# Autodesk Inventor assembly: Application_openUC2_QBox_2
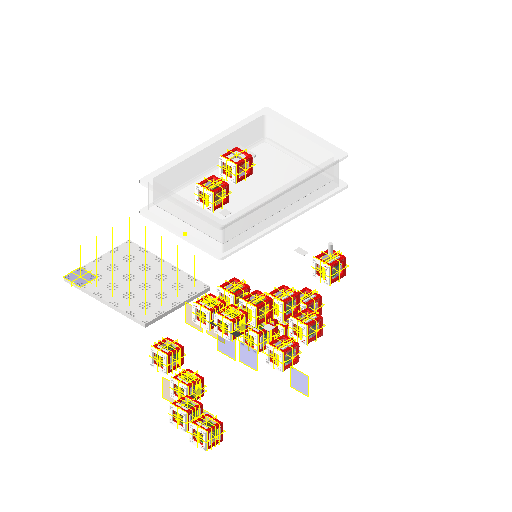
[picture p0: Inventor's stored thumbnail of the model, 512x512]
Saved by Autodesk Inventor 2025.1 (Build 291241020, 241B)
## iProperties
Created: 2022-07-25
Part Number: Application_openUC2_QBox_2
Document SubType Name: Assembly
Designer: diederichbenedict
Mass: 3359.27 g
Surface Area: 10315 cm^2
Volume: 3354.93 cm^3
Density: 1.00129 g/cm^3
Author: diederichbenedict
## Documents named in this file (12)
- C:\Users\diederichbenedict\Dropbox\Dokumente\Promotion\PROJECTS\TechnicalDocs-openUC2-QBox\Production_Files\CAD_Files\INVENTOR\Application_openUC2_QBox_2.iam
- C:\Users\diederichbenedict\Dropbox\Dokumente\Promotion\PROJECTS\TechnicalDocs-openUC2-QBox\Production_Files\CAD_Files\INVENTOR\00_Really_Useful_Box_4l_DinA4_body.ipt
- C:\Users\diederichbenedict\Dropbox\Dokumente\Promotion\PROJECTS\TechnicalDocs-openUC2-QBox\Production_Files\CAD_Files\INVENTOR\Assembly_Cube_v4_Beamsplittercube_20mm.iam
- C:\Users\diederichbenedict\Dropbox\Dokumente\Promotion\PROJECTS\TechnicalDocs-openUC2-QBox\Production_Files\CAD_Files\INVENTOR\Assembly_Cube_v4_Lens.iam
- C:\Users\diederichbenedict\Dropbox\Dokumente\Promotion\PROJECTS\TechnicalDocs-openUC2-QBox\Production_Files\CAD_Files\INVENTOR\Assembly_Cube_v4_KinematicMirror_45°.iam
- C:\Users\diederichbenedict\Dropbox\Dokumente\Promotion\PROJECTS\TechnicalDocs-openUC2-QBox\Production_Files\CAD_Files\INVENTOR\Assembly_Cube_v4_Photosensor.iam
- C:\Users\diederichbenedict\Dropbox\Dokumente\Promotion\PROJECTS\TechnicalDocs-openUC2-QBox\Production_Files\CAD_Files\INVENTOR\Assembly_Cube_v4_polfilter.iam
- C:\Users\diederichbenedict\Dropbox\Dokumente\Promotion\PROJECTS\TechnicalDocs-openUC2-QBox\Production_Files\CAD_Files\INVENTOR\Assembly_Cube_v4_magnet_tshirt.iam
- C:\Users\diederichbenedict\Dropbox\Dokumente\Promotion\PROJECTS\TechnicalDocs-openUC2-QBox\Production_Files\CAD_Files\INVENTOR\Assembly_Cube_v4_slideframe_holder.iam
- C:\Users\diederichbenedict\Dropbox\Dokumente\Promotion\PROJECTS\TechnicalDocs-openUC2-QBox\Production_Files\CAD_Files\INVENTOR\Assembly_Cube_v4_xystage_diamond.iam
- C:\Users\diederichbenedict\Dropbox\Dokumente\Promotion\PROJECTS\TechnicalDocs-openUC2-QBox\Production_Files\CAD_Files\INVENTOR\20_Baseplate_POM_10mm.ipt
- C:\Users\diederichbenedict\Dropbox\Dokumente\Promotion\PROJECTS\TechnicalDocs-openUC2-QBox\Production_Files\CAD_Files\INVENTOR\Assembly_Cube_v4_Laser_v4.iam
## Components (20 placed, 11 different names)
1. 00_Really_Useful_Box_4l_DinA4_body:1 — Mate:12
2. Assembly_Cube_v4_Beamsplittercube_20mm:1 [sub-assembly]
3. Assembly_Cube_v4_Beamsplittercube_20mm:2 [sub-assembly]
4. Assembly_Cube_v4_Beamsplittercube_20mm:4 [sub-assembly]
5. Assembly_Cube_v4_Beamsplittercube_20mm:3 [sub-assembly]
6. Assembly_Cube_v4_KinematicMirror_45°:1 [sub-assembly]
7. Assembly_Cube_v4_KinematicMirror_45°:2 [sub-assembly]
8. Assembly_Cube_v4_KinematicMirror_45°:3 [sub-assembly]
9. Assembly_Cube_v4_polfilter:1 [sub-assembly]
10. Assembly_Cube_v4_polfilter:2 [sub-assembly]
11. Assembly_Cube_v4_magnet_tshirt:1 [sub-assembly]
12. Assembly_Cube_v4_Lens:1 [sub-assembly]
13. Assembly_Cube_v4_Lens:2 [sub-assembly]
14. Assembly_Cube_v4_Lens:3 [sub-assembly]
15. Assembly_Cube_v4_Photosensor:1 [sub-assembly]
16. Assembly_Cube_v4_slideframe_holder:1 [sub-assembly]
17. Assembly_Cube_v4_xystage_diamond:1 [sub-assembly]
18. Assembly_Cube_v4_polfilter:3 [sub-assembly]
19. 20_Baseplate_POM_10mm:1
20. Assembly_Cube_v4_Laser_v4:1 [sub-assembly]
## Relationships (1: Mate 1)
- Mate:12: 00_Really_Useful_Box_4l_DinA4_body:1
